# Autodesk Inventor assembly: iris
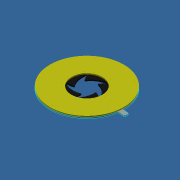
[picture p0: Inventor's stored thumbnail of the model, 180x180]
Saved by Autodesk Inventor 2014 (Build 180170000, 170)
## iProperties
Created: 2014-03-15
Part Number: iris
Document SubType Name: Assembly
Designer: Lefo
Author: Lefo
## Documents named in this file (5)
- C:\Users\Lefo\Documents\Inventor\academy\something big\iris.iam
- C:\Users\Lefo\Documents\Inventor\academy\something big\plancha.ipt
- C:\Users\Lefo\Documents\Inventor\academy\petalo3.ipt
- C:\Users\Lefo\Documents\Inventor\academy\borde.ipt
- C:\Users\Lefo\Documents\Inventor\academy\brazo.ipt
## Components (12 placed, 4 different names)
1. plancha:1 — Insert:1, Insert:2, Insert:3, Insert:4, Insert:5, Flush:1, Mate:1, Flush:2
2. petalo3:1 — Insert:1, Insert:18
3. petalo3:2 — Insert:3, Insert:16
4. petalo3:3 — Insert:2, Insert:10
5. petalo3:4 — Insert:4, Insert:14
6. petalo3:5 — Insert:5, Insert:12
7. borde:1 — Flush:1, Insert:9, Mate:1, Insert:11, Insert:13, Insert:15, Insert:17, Flush:2
8. brazo:1 — Insert:9, Insert:10
9. brazo:2 — Insert:17, Insert:18
10. brazo:3 — Insert:15, Insert:16
11. brazo:4 — Insert:13, Insert:14
12. brazo:5 — Insert:11, Insert:12
## Relationships (18: Insert 15, Flush 2, Mate 1)
- Insert:1: plancha:1 ↔ petalo3:1
- Insert:2: plancha:1 ↔ petalo3:3
- Insert:3: plancha:1 ↔ petalo3:2
- Insert:4: plancha:1 ↔ petalo3:4
- Insert:5: plancha:1 ↔ petalo3:5
- Flush:1: plancha:1 ↔ borde:1
- Insert:9: borde:1 ↔ brazo:1
- Insert:10: petalo3:3 ↔ brazo:1
- Mate:1: plancha:1 ↔ borde:1
- Insert:11: borde:1 ↔ brazo:5
- Insert:12: petalo3:5 ↔ brazo:5
- Insert:13: borde:1 ↔ brazo:4
- Insert:14: petalo3:4 ↔ brazo:4
- Insert:15: borde:1 ↔ brazo:3
- Insert:16: petalo3:2 ↔ brazo:3
- Insert:17: borde:1 ↔ brazo:2
- Insert:18: petalo3:1 ↔ brazo:2
- Flush:2: plancha:1 ↔ borde:1
